# Autodesk Inventor assembly: Assembly1
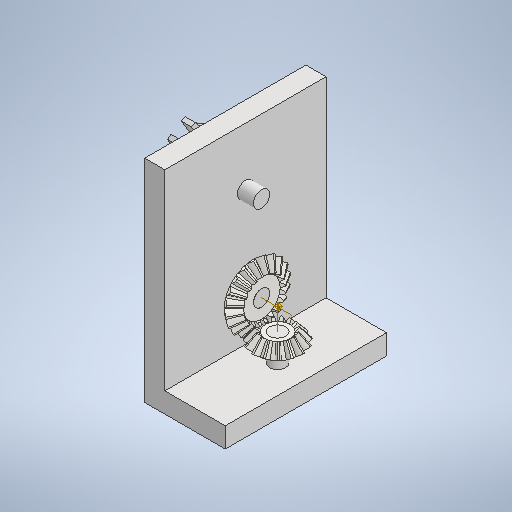
[picture p0: Inventor's stored thumbnail of the model, 512x512]
Saved by Autodesk Inventor 2025.2 (Build 292293000, 293)
## iProperties
Created: 2025-01-23
Part Number: Assembly1
Document SubType Name: Assembly
Designer: yash3
Author: yash3
## Documents named in this file (9)
- C:\Users\yash3\Documents\ta212\Assembly1.iam
- C:\Users\yash3\Documents\ta212\Support_Plate.ipt
- C:\Users\yash3\Documents\ta212\Geneva_driver.ipt
- C:\Users\yash3\Documents\ta212\Geneva_driven.ipt
- C:\Users\yash3\Documents\ta212\Shaft.ipt
- C:\Users\yash3\Documents\ta212\Assembly1\Design Accelerator\Bevel Gears1.iam
- C:\Users\yash3\Documents\ta212\Assembly1\Design Accelerator\Bevel Gears3.iam
- C:\Users\yash3\Documents\ta212\Assembly1\Design Accelerator\Bevel Gears4.iam
- C:\Users\yash3\Documents\ta212\Assembly1\Design Accelerator\Bevel Gears5.iam
## Components (10 placed, 5 different names)
1. Support_Plate:1 — Mate:1, Mate:2, Mate:4, Mate:9
2. Geneva_driver:1 — Mate:1, Mate:2, Mate:3, Mate:7, Mate:8, Rotation:4
3. Geneva_driven:1 — Mate:3, Mate:4, Mate:5, Mate:6
4. Shaft:1 — Mate:5, Mate:6
5. Shaft:2 — Mate:7, Mate:8, Mate:10, Rotation:3, Rotation:4
6. Shaft:3 — Mate:9, Mate:11, Flush:1, Rotation:2
7. Bevel Gears:1 [sub-assembly]
8. Bevel Gears:2 [sub-assembly]
9. Bevel Gears:3 [sub-assembly] — Mate:10, Mate:12, Rotation:1, Rotation:3
10. Bevel Gears:4 [sub-assembly] — Mate:11, Mate:12, Flush:1, Rotation:1, Rotation:2
## Relationships (17: Mate 12, RelateRotation 4, Flush 1)
- Mate:1: Support_Plate:1 ↔ Geneva_driver:1
- Mate:2: Support_Plate:1 ↔ Geneva_driver:1
- Mate:3: Geneva_driver:1 ↔ Geneva_driven:1
- Mate:4: Support_Plate:1 ↔ Geneva_driven:1
- Mate:5: Geneva_driven:1 ↔ Shaft:1
- Mate:6: Geneva_driven:1 ↔ Shaft:1
- Mate:7: Geneva_driver:1 ↔ Shaft:2
- Mate:8: Geneva_driver:1 ↔ Shaft:2
- Mate:9: Support_Plate:1 ↔ Shaft:3
- Mate:10: Shaft:2 ↔ Bevel Gears:3
- Mate:11: Shaft:3 ↔ Bevel Gears:4
- Mate:12: Bevel Gears:3 ↔ Bevel Gears:4
- Flush:1: Shaft:3 ↔ Bevel Gears:4
- Rotation:1 [RelateRotation] (1.3333 ul): Bevel Gears:3 ↔ Bevel Gears:4
- Rotation:2 [RelateRotation] (1 ul): Shaft:3 ↔ Bevel Gears:4
- Rotation:3 [RelateRotation] (1 ul): Shaft:2 ↔ Bevel Gears:3
- Rotation:4 [RelateRotation] (1 ul): Geneva_driver:1 ↔ Shaft:2
